# Autodesk Inventor assembly: teljes3
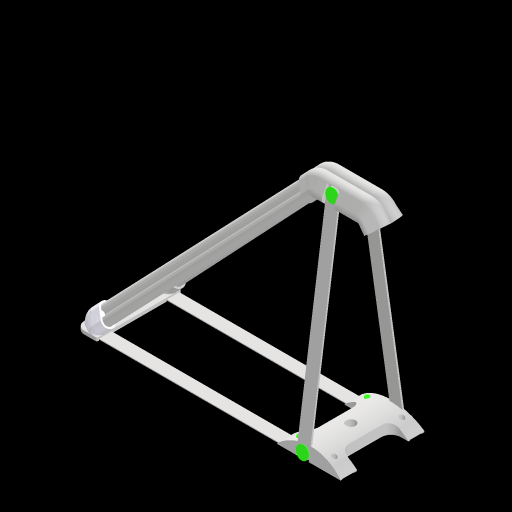
[picture p0: Inventor's stored thumbnail of the model, 512x512]
Saved by Autodesk Inventor 2023 (Build 270158000, 158)
## iProperties
Created: 2022-11-11
Part Number: teljes3
Document SubType Name: Assembly
Designer: gd1
Author: gd1
## Documents named in this file (9)
- C:\Users\gd1\3D Objects\3D nagyteherbírású híd\Híd\H-d\teljes4.iam
- C:\Users\gd1\3D Objects\3D nagyteherbírású híd\Híd\H-d\45 fok középre.ipt
- C:\Users\gd1\3D Objects\3D nagyteherbírású híd\Híd\H-d\palca 325mm.ipt
- C:\Users\gd1\3D Objects\3D nagyteherbírású híd\Híd\H-d\kozepso szalag2.ipt
- C:\Users\gd1\3D Objects\3D nagyteherbírású híd\Híd\H-d\45 fok kozepcsati.ipt.iam
- C:\Users\gd1\3D Objects\3D nagyteherbírású híd\Híd\H-d\közepső szalag 1.ipt
- C:\Users\gd1\3D Objects\3D nagyteherbírású híd\Híd\H-d\kozepso_csomopont.ipt
- C:\Users\gd1\3D Objects\3D nagyteherbírású híd\Híd\H-d\tipli.ipt
- 45 fok kozepcsati.ipt
## Components (17 placed, 7 different names)
1. 45 fok középre:1 — Rotational:1, Rotational:2, Rotational:7, Rotational:8
2. palca 325mm:1 — Rotational:2
3. palca 325mm:2 — Rotational:1
4. 45 fok kozepcsati.ipt:1 [sub-assembly] — Rigid:2, Rotational:10
5. közepső szalag 1:1 — Rigid:2, Rigid:4, Rotational:13
6. közepső szalag 1:2 — Rotational:10, Rotational:14, Rotational:15
7. kozepso szalag2:1 — Rotational:7, Rotational:9, Rotational:11, Rotational:12
8. kozepso szalag2:2 — Rotational:8, Rigid:3, Rotational:16
9. kozepso_csomopont:1 — Rotational:9
10. tipli:1 — Rotational:16
11. tipli:2 — Rotational:13
12. tipli:3 — Rotational:15
13. tipli:4 — Rotational:12
14. tipli:5 — Rotational:11
15. tipli:6 — Rigid:3
16. tipli:7 — Rigid:4
17. tipli:8 — Rotational:14
## Relationships (15: RevoluteJoint 12, WeldJoint 3)
- Rotational:1 [RevoluteJoint]: 45 fok középre:1 ↔ palca 325mm:2
- Rotational:2 [RevoluteJoint]: 45 fok középre:1 ↔ palca 325mm:1
- Rotational:7 [RevoluteJoint]: 45 fok középre:1 ↔ kozepso szalag2:1
- Rotational:8 [RevoluteJoint]: 45 fok középre:1 ↔ kozepso szalag2:2
- Rigid:2 [WeldJoint]: 45 fok kozepcsati.ipt:1 ↔ közepső szalag 1:1
- Rotational:9 [RevoluteJoint]: kozepso szalag2:1 ↔ kozepso_csomopont:1
- Rotational:10 [RevoluteJoint]: 45 fok kozepcsati.ipt:1 ↔ közepső szalag 1:2
- Rotational:11 [RevoluteJoint]: kozepso szalag2:1 ↔ tipli:5
- Rigid:3 [WeldJoint]: kozepso szalag2:2 ↔ tipli:6
- Rigid:4 [WeldJoint]: közepső szalag 1:1 ↔ tipli:7
- Rotational:12 [RevoluteJoint]: kozepso szalag2:1 ↔ tipli:4
- Rotational:13 [RevoluteJoint]: közepső szalag 1:1 ↔ tipli:2
- Rotational:14 [RevoluteJoint]: közepső szalag 1:2 ↔ tipli:8
- Rotational:15 [RevoluteJoint]: közepső szalag 1:2 ↔ tipli:3
- Rotational:16 [RevoluteJoint]: kozepso szalag2:2 ↔ tipli:1
